# Autodesk Inventor assembly: Grundplatte_test
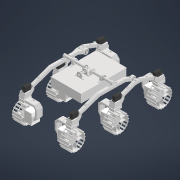
[picture p0: Inventor's stored thumbnail of the model, 180x180]
Saved by Autodesk Inventor 2021 (Build 250183000, 183)
## iProperties
Created: 2021-01-26
Part Number: Grundplatte_test
Document SubType Name: Assembly
Designer: Ctroi
Author: Ctroi
## Documents named in this file (33)
- G:\Roverprojekt\Github Projekt\Rover\Grundplatte_test.iam
- G:\Roverprojekt\Github Projekt\Rover\Grundplatte_hinten.ipt
- G:\Roverprojekt\Github Projekt\Rover\Grundplatte_vorne.ipt
- G:\Roverprojekt\Github Projekt\Rover\ArduinoMega.ipt
- G:\Roverprojekt\Github Projekt\Rover\Relais.ipt
- G:\Roverprojekt\Github Projekt\Rover\Kreuz_Halterung.ipt
- G:\Roverprojekt\Github Projekt\Rover\Obenplatte_hinten.ipt
- G:\Roverprojekt\Github Projekt\Rover\Obenplatte_vorne.ipt
- G:\Roverprojekt\Github Projekt\Rover\Halterung_Differential_3.ipt
- G:\Roverprojekt\Github Projekt\Rover\Halterung_Differential_Mitte.ipt
- G:\Roverprojekt\Github Projekt\Rover\Halterung_Differential.ipt
- G:\Roverprojekt\Github Projekt\Rover\Halterung_Differential_2.ipt
- G:\Roverprojekt\Github Projekt\Rover\Kugellager.ipt
- G:\Roverprojekt\Github Projekt\Rover\Kugellager_klein.ipt
- G:\Roverprojekt\Github Projekt\Rover\Verbindung_Rocker_Body.ipt
- G:\Roverprojekt\Github Projekt\Rover\Welle_Kugellager_Mitte.ipt
- G:\Roverprojekt\Github Projekt\Rover\Rocker_hinten_rechts.ipt
- G:\Roverprojekt\Github Projekt\Rover\Rocker_hinten.ipt
- G:\Roverprojekt\Github Projekt\Rover\Rocker_vorne.ipt
- G:\Roverprojekt\Github Projekt\Rover\Bogie.ipt
- G:\Roverprojekt\Github Projekt\Rover\Boogie_Stange.ipt
- G:\Roverprojekt\Github Projekt\Rover\Servohalterung_v2.ipt
- G:\Roverprojekt\Github Projekt\Rover\Servo.ipt
- G:\Roverprojekt\Github Projekt\Rover\Gegenstück_Welle_Diff.ipt
- G:\Roverprojekt\Github Projekt\Rover\Zahnrad_innen.ipt
- G:\Roverprojekt\Github Projekt\Rover\Übersetzungsbox_2.ipt
- G:\Roverprojekt\Github Projekt\Rover\Zahnrad_außen.ipt
- G:\Roverprojekt\Github Projekt\Rover\Motor_Servo_Welle_Test.ipt
- G:\Roverprojekt\Github Projekt\Rover\Verbindung_Motor_Servo_v2.ipt
- G:\Roverprojekt\Github Projekt\Rover\Motorhalterung_Klemme.ipt
- G:\Roverprojekt\Github Projekt\Rover\Motorhalterung_v2.ipt
- G:\Roverprojekt\Github Projekt\Rover\Steppermotor.ipt
- G:\Roverprojekt\Github Projekt\Rover\Reifen_v2.ipt
## Components (107 placed, 31 different names)
1. Grundplatte_hinten:1 — Passend:1, Passend:2, Passend:5, Passend:6, Passend:7, Passend:11, Passend:12, Passend:13, Passend:16
2. Grundplatte_vorne:1 — Passend:1, Passend:2, Passend:3, Passend:4, Passend:8, Passend:9, Passend:10, Passend:16
3. ArduinoMega:1 — Passend:3, Passend:4
4. Relais:1
5. Kreuz_Halterung:1 — Passend:5, Passend:6, Passend:7
6. Gegenstück_Welle_Diff:1 — Passend:96, Passend:97
7. Welle_Kugellager_Mitte:1 — Passend:48, Passend:49, Passend:96, Passend:97
8. Obenplatte_vorne:1 — Passend:8, Passend:9, Passend:10, Passend:15, Passend:17, Passend:18, Passend:21, Passend:22, Passend:23, Passend:24, Passend:27, Passend:28
9. Halterung_Differential_3:1 — Passend:14, Passend:15, Passend:17, Passend:38, Passend:39
10. Halterung_Differential_3:2 — Passend:18, Passend:19, Passend:20, Passend:32, Passend:33
11. Obenplatte_hinten:1 — Passend:11, Passend:12, Passend:13, Passend:14, Passend:19, Passend:20, Passend:25, Passend:26
12. Halterung_Differential_Mitte:1 — Passend:21, Passend:22, Passend:23, Passend:42, Passend:43
13. Halterung_Differential:1 — Passend:26, Passend:27, Passend:28, Passend:30, Passend:31, Passend:36, Passend:37
14. Halterung_Differential:2 — Passend:24, Passend:25, Passend:29, Passend:34, Passend:35
15. Halterung_Differential_2:1 — Passend:29, Passend:30, Passend:31, Passend:40, Passend:41
16. Kugellager:1 — Passend:40, Passend:41, Passend:48, Passend:49
17. Kugellager:2 — Passend:32, Passend:33, Passend:47
18. Kugellager:3 — Passend:34, Passend:35, Passend:44
19. Kugellager:4 — Passend:36, Passend:37, Passend:45
20. Kugellager:5 — Passend:38, Passend:39, Passend:46
21. Kugellager_klein:1 — Passend:42, Passend:43
22. Reifen_v2:6 — Einfügen:3
23. Reifen_v2:5 — Einfügen:4
24. Reifen_v2:4 — Einfügen:5
25. Steppermotor:6 — Passend:191, Passend:192, Passend:193, Einfügen:5
26. Steppermotor:5 — Passend:188, Passend:189, Passend:190, Einfügen:4
27. Steppermotor:4 — Passend:185, Passend:186, Passend:187, Einfügen:3
28. Motorhalterung_v2:3 — Fluchtend:41, Fluchtend:42, Passend:170, Passend:185, Passend:186, Passend:187
29. Motorhalterung_v2:2 — Fluchtend:43, Fluchtend:44, Passend:171, Passend:188, Passend:189, Passend:190
30. Motorhalterung_v2:1 — Fluchtend:45, Fluchtend:46, Passend:172, Passend:191, Passend:192, Passend:193
31. Motorhalterung_Klemme:3 — Fluchtend:33, Fluchtend:34, Passend:166, Fluchtend:45, Fluchtend:46, Passend:172
32. Motorhalterung_Klemme:2 — Fluchtend:31, Fluchtend:32, Passend:165, Fluchtend:43, Fluchtend:44, Passend:171
33. Motorhalterung_Klemme:1 — Fluchtend:29, Fluchtend:30, Passend:164, Fluchtend:41, Fluchtend:42, Passend:170
34. Verbindung_Motor_Servo_v2:6 — Passend:158, Passend:159, Fluchtend:29, Fluchtend:30, Passend:164
35. Verbindung_Motor_Servo_v2:5 — Passend:162, Passend:163, Fluchtend:33, Fluchtend:34, Passend:166
36. Verbindung_Motor_Servo_v2:4 — Passend:160, Passend:161, Fluchtend:31, Fluchtend:32, Passend:165
37. Motor_Servo_Welle_Test:6 — Passend:150, Passend:151, Passend:158, Passend:159
38. Motor_Servo_Welle_Test:5 — Passend:148, Passend:149, Passend:162, Passend:163
39. Motor_Servo_Welle_Test:4 — Passend:146, Passend:147, Passend:160, Passend:161
40. Zahnrad_außen:6 — Passend:136, Passend:137
41. Zahnrad_außen:5 — Passend:138, Passend:139
42. Zahnrad_außen:4 — Passend:134, Passend:135
43. Kugellager:14 — Passend:122, Passend:123, Passend:148, Passend:149
44. Kugellager:13 — Passend:124, Passend:125, Passend:146, Passend:147
45. Kugellager:10 — Passend:126, Passend:127, Passend:150, Passend:151
46. Übersetzungsbox_2:6 — Fluchtend:25, Fluchtend:26, Passend:114, Passend:124, Passend:125
47. Übersetzungsbox_2:3 — Fluchtend:27, Fluchtend:28, Passend:115, Passend:122, Passend:123
48. Übersetzungsbox_2:2 — Fluchtend:19, Fluchtend:20, Passend:111, Passend:126, Passend:127
49. Zahnrad_innen:3 — Passend:102, Passend:103, Passend:136, Passend:137
50. Zahnrad_innen:2 — Passend:100, Passend:101, Passend:138, Passend:139
51. Zahnrad_innen:1 — Passend:98, Passend:99, Passend:134, Passend:135
52. Servo:3 — Passend:81, Passend:82, Passend:83, Passend:102, Passend:103
53. Servo:5 — Passend:93, Passend:94, Passend:95, Passend:100, Passend:101
54. Servo:2 — Passend:90, Passend:91, Passend:92, Passend:98, Passend:99
55. Servohalterung_v2:5 — Fluchtend:15, Fluchtend:16, Passend:77, Passend:90, Passend:91, Passend:92, Fluchtend:19, Fluchtend:20, Passend:111
56. Servohalterung_v2:3 — Fluchtend:13, Fluchtend:14, Passend:76, Passend:93, Passend:94, Passend:95, Fluchtend:25, Fluchtend:26, Passend:114
57. Servohalterung_v2:2 — Fluchtend:11, Fluchtend:12, Passend:75, Passend:81, Passend:82, Passend:83, Fluchtend:27, Fluchtend:28, Passend:115
58. Boogie_Stange:1 — Passend:64, Passend:65, Passend:68, Passend:69
59. Fahrwerk_bogie:2 — Passend:68, Passend:69, Fluchtend:13, Fluchtend:14, Passend:76, Fluchtend:15, Fluchtend:16, Passend:77
60. Fahrwerk_rocker_vorne:1 — Fluchtend:1, Fluchtend:2, Passend:62, Fluchtend:11, Fluchtend:12, Passend:75
61. Kugellager:7 — Passend:54, Passend:55, Passend:64, Passend:65
62. Kugellager:6 — Passend:52, Passend:53
63. Fahrwerk_rocker_hinten:1 — Passend:50, Passend:51, Passend:52, Passend:53, Passend:54, Passend:55, Fluchtend:1, Fluchtend:2, Passend:62
64. Verbindung_Rocker_Body:1 — Passend:44, Passend:47, Passend:50, Passend:51
65. Reifen_v2:3 — Einfügen:2
66. Reifen_v2:2 — Einfügen:1
67. Reifen_v2:1
68. Steppermotor:3 — Passend:182, Passend:183, Passend:184
69. Steppermotor:2 — Passend:179, Passend:180, Passend:181, Einfügen:2
70. Steppermotor:1 — Passend:176, Passend:177, Passend:178, Einfügen:1
71. Motorhalterung_v2:6 — Fluchtend:51, Fluchtend:52, Passend:175, Passend:182, Passend:183, Passend:184
72. Motorhalterung_v2:5 — Fluchtend:49, Fluchtend:50, Passend:174, Passend:179, Passend:180, Passend:181
73. Motorhalterung_v2:4 — Fluchtend:47, Fluchtend:48, Passend:173, Passend:176, Passend:177, Passend:178
74. Motorhalterung_Klemme:4 — Fluchtend:35, Fluchtend:36, Passend:167, Fluchtend:47, Fluchtend:48, Passend:173
75. Motorhalterung_Klemme:5 — Fluchtend:37, Fluchtend:38, Passend:168, Fluchtend:49, Fluchtend:50, Passend:174
76. Motorhalterung_Klemme:6 — Fluchtend:39, Fluchtend:40, Passend:169, Fluchtend:51, Fluchtend:52, Passend:175
77. Verbindung_Motor_Servo_v2:3 — Passend:152, Passend:153, Fluchtend:35, Fluchtend:36, Passend:167
78. Verbindung_Motor_Servo_v2:2 — Passend:156, Passend:157, Fluchtend:39, Fluchtend:40, Passend:169
79. Verbindung_Motor_Servo_v2:1 — Passend:154, Passend:155, Fluchtend:37, Fluchtend:38, Passend:168
80. Motor_Servo_Welle_Test:3 — Passend:144, Passend:145, Passend:156, Passend:157
81. Motor_Servo_Welle_Test:2 — Passend:140, Passend:141, Passend:152, Passend:153
82. Motor_Servo_Welle_Test:1 — Passend:142, Passend:143, Passend:154, Passend:155
83. Zahnrad_außen:3 — Passend:132, Passend:133
84. Zahnrad_außen:2 — Passend:130, Passend:131
85. Zahnrad_außen:1 — Passend:128, Passend:129
86. Kugellager:15 — Passend:120, Passend:121, Passend:140, Passend:141
87. Kugellager:12 — Passend:118, Passend:119, Passend:142, Passend:143
88. Kugellager:11 — Passend:116, Passend:117, Passend:144, Passend:145
89. Übersetzungsbox_2:5 — Fluchtend:21, Fluchtend:22, Passend:112, Passend:118, Passend:119
90. Übersetzungsbox_2:4 — Fluchtend:23, Fluchtend:24, Passend:113, Passend:120, Passend:121
91. Übersetzungsbox_2:1 — Fluchtend:17, Fluchtend:18, Passend:110, Passend:116, Passend:117
92. Zahnrad_innen:6 — Passend:108, Passend:109, Passend:132, Passend:133
93. Zahnrad_innen:5 — Passend:106, Passend:107, Passend:130, Passend:131
94. Zahnrad_innen:4 — Passend:104, Passend:105, Passend:128, Passend:129
95. Servo:4 — Passend:78, Passend:79, Passend:80, Passend:108, Passend:109
96. Servo:6 — Passend:84, Passend:85, Passend:86, Passend:106, Passend:107
97. Servo:1 — Passend:87, Passend:88, Passend:89, Passend:104, Passend:105
98. Servohalterung_v2:6 — Fluchtend:5, Fluchtend:6, Passend:72, Passend:87, Passend:88, Passend:89, Fluchtend:17, Fluchtend:18, Passend:110
99. Servohalterung_v2:4 — Fluchtend:7, Fluchtend:8, Passend:73, Passend:84, Passend:85, Passend:86, Fluchtend:21, Fluchtend:22, Passend:112
100. Servohalterung_v2:1 — Fluchtend:9, Fluchtend:10, Passend:74, Passend:78, Passend:79, Passend:80, Fluchtend:23, Fluchtend:24, Passend:113
101. Boogie_Stange:2 — Passend:66, Passend:67, Passend:70, Passend:71
102. Fahrwerk_bogie:1 — Passend:70, Passend:71, Fluchtend:5, Fluchtend:6, Passend:72, Fluchtend:7, Fluchtend:8, Passend:73
103. Kugellager:9 — Passend:60, Passend:61
104. Kugellager:8 — Passend:58, Passend:59, Passend:66, Passend:67
105. Fahrwerk_rocker_hinten:2 — Passend:56, Passend:57, Passend:58, Passend:59, Passend:60, Passend:61, Fluchtend:3, Fluchtend:4, Passend:63
106. Fahrwerk_rocker_vorne:2 — Fluchtend:3, Fluchtend:4, Passend:63, Fluchtend:9, Fluchtend:10, Passend:74
107. Verbindung_Rocker_Body:2 — Passend:45, Passend:46, Passend:56, Passend:57
## Relationships (250: Mate 193, Flush 52, Insert 5)
- Passend:1 [Mate]: Grundplatte_hinten:1 ↔ Grundplatte_vorne:1
- Passend:2 [Mate]: Grundplatte_hinten:1 ↔ Grundplatte_vorne:1
- Passend:3 [Mate]: Grundplatte_vorne:1 ↔ ArduinoMega:1
- Passend:4 [Mate]: Grundplatte_vorne:1 ↔ ArduinoMega:1
- Passend:5 [Mate]: Grundplatte_hinten:1 ↔ Kreuz_Halterung:1
- Passend:6 [Mate]: Grundplatte_hinten:1 ↔ Kreuz_Halterung:1
- Passend:7 [Mate]: Grundplatte_hinten:1 ↔ Kreuz_Halterung:1
- Passend:8 [Mate]: Grundplatte_vorne:1 ↔ Obenplatte_vorne:1
- Passend:9 [Mate]: Grundplatte_vorne:1 ↔ Obenplatte_vorne:1
- Passend:10 [Mate]: Grundplatte_vorne:1 ↔ Obenplatte_vorne:1
- Passend:11 [Mate]: Grundplatte_hinten:1 ↔ Obenplatte_hinten:1
- Passend:12 [Mate]: Grundplatte_hinten:1 ↔ Obenplatte_hinten:1
- Passend:13 [Mate]: Grundplatte_hinten:1 ↔ Obenplatte_hinten:1
- Passend:14 [Mate]: Halterung_Differential_3:1 ↔ Obenplatte_hinten:1
- Passend:15 [Mate]: Obenplatte_vorne:1 ↔ Halterung_Differential_3:1
- Passend:16 [Mate]: Grundplatte_hinten:1 ↔ Grundplatte_vorne:1
- Passend:17 [Mate]: Obenplatte_vorne:1 ↔ Halterung_Differential_3:1
- Passend:18 [Mate]: Obenplatte_vorne:1 ↔ Halterung_Differential_3:2
- Passend:19 [Mate]: Halterung_Differential_3:2 ↔ Obenplatte_hinten:1
- Passend:20 [Mate]: Halterung_Differential_3:2 ↔ Obenplatte_hinten:1
- Passend:21 [Mate]: Obenplatte_vorne:1 ↔ Halterung_Differential_Mitte:1
- Passend:22 [Mate]: Obenplatte_vorne:1 ↔ Halterung_Differential_Mitte:1
- Passend:23 [Mate]: Obenplatte_vorne:1 ↔ Halterung_Differential_Mitte:1
- Passend:24 [Mate]: Obenplatte_vorne:1 ↔ Halterung_Differential:2
- Passend:25 [Mate]: Obenplatte_hinten:1 ↔ Halterung_Differential:2
- Passend:26 [Mate]: Obenplatte_hinten:1 ↔ Halterung_Differential:1
- Passend:27 [Mate]: Obenplatte_vorne:1 ↔ Halterung_Differential:1
- Passend:28 [Mate]: Obenplatte_vorne:1 ↔ Halterung_Differential:1
- Passend:29 [Mate]: Halterung_Differential:2 ↔ Halterung_Differential_2:1
- Passend:30 [Mate]: Halterung_Differential:1 ↔ Halterung_Differential_2:1
- Passend:31 [Mate]: Halterung_Differential:1 ↔ Halterung_Differential_2:1
- Passend:32 [Mate]: Halterung_Differential_3:2 ↔ Kugellager:2
- Passend:33 [Mate]: Halterung_Differential_3:2 ↔ Kugellager:2
- Passend:34 [Mate]: Halterung_Differential:2 ↔ Kugellager:3
- Passend:35 [Mate]: Halterung_Differential:2 ↔ Kugellager:3
- Passend:36 [Mate]: Halterung_Differential:1 ↔ Kugellager:4
- Passend:37 [Mate]: Halterung_Differential:1 ↔ Kugellager:4
- Passend:38 [Mate]: Halterung_Differential_3:1 ↔ Kugellager:5
- Passend:39 [Mate]: Halterung_Differential_3:1 ↔ Kugellager:5
- Passend:40 [Mate]: Halterung_Differential_2:1 ↔ Kugellager:1
- Passend:41 [Mate]: Halterung_Differential_2:1 ↔ Kugellager:1
- Passend:42 [Mate]: Halterung_Differential_Mitte:1 ↔ Kugellager_klein:1
- Passend:43 [Mate]: Halterung_Differential_Mitte:1 ↔ Kugellager_klein:1
- Passend:44 [Mate]: Kugellager:3 ↔ Verbindung_Rocker_Body:1
- Passend:45 [Mate]: Kugellager:4 ↔ Verbindung_Rocker_Body:2
- Passend:46 [Mate]: Kugellager:5 ↔ Verbindung_Rocker_Body:2
- Passend:47 [Mate]: Kugellager:2 ↔ Verbindung_Rocker_Body:1
- Passend:48 [Mate]: Welle_Kugellager_Mitte:1 ↔ Kugellager:1
- Passend:49 [Mate]: Welle_Kugellager_Mitte:1 ↔ Kugellager:1
- Passend:50 [Mate]: Fahrwerk_rocker_hinten:1 ↔ Verbindung_Rocker_Body:1
- Passend:51 [Mate]: Fahrwerk_rocker_hinten:1 ↔ Verbindung_Rocker_Body:1
- Passend:52 [Mate]: Kugellager:6 ↔ Fahrwerk_rocker_hinten:1
- Passend:53 [Mate]: Kugellager:6 ↔ Fahrwerk_rocker_hinten:1
- Passend:54 [Mate]: Kugellager:7 ↔ Fahrwerk_rocker_hinten:1
- Passend:55 [Mate]: Kugellager:7 ↔ Fahrwerk_rocker_hinten:1
- Passend:56 [Mate]: Fahrwerk_rocker_hinten:2 ↔ Verbindung_Rocker_Body:2
- Passend:57 [Mate]: Fahrwerk_rocker_hinten:2 ↔ Verbindung_Rocker_Body:2
- Passend:58 [Mate]: Kugellager:8 ↔ Fahrwerk_rocker_hinten:2
- Passend:59 [Mate]: Kugellager:8 ↔ Fahrwerk_rocker_hinten:2
- Passend:60 [Mate]: Kugellager:9 ↔ Fahrwerk_rocker_hinten:2
- Passend:61 [Mate]: Kugellager:9 ↔ Fahrwerk_rocker_hinten:2
- Fluchtend:1 [Flush]: Fahrwerk_rocker_vorne:1 ↔ Fahrwerk_rocker_hinten:1
- Fluchtend:2 [Flush]: Fahrwerk_rocker_vorne:1 ↔ Fahrwerk_rocker_hinten:1
- Passend:62 [Mate]: Fahrwerk_rocker_vorne:1 ↔ Fahrwerk_rocker_hinten:1
- Fluchtend:3 [Flush]: Fahrwerk_rocker_hinten:2 ↔ Fahrwerk_rocker_vorne:2
- Fluchtend:4 [Flush]: Fahrwerk_rocker_hinten:2 ↔ Fahrwerk_rocker_vorne:2
- Passend:63 [Mate]: Fahrwerk_rocker_hinten:2 ↔ Fahrwerk_rocker_vorne:2
- Passend:64 [Mate]: Boogie_Stange:1 ↔ Kugellager:7
- Passend:65 [Mate]: Boogie_Stange:1 ↔ Kugellager:7
- Passend:66 [Mate]: Boogie_Stange:2 ↔ Kugellager:8
- Passend:67 [Mate]: Boogie_Stange:2 ↔ Kugellager:8
- Passend:68 [Mate]: Boogie_Stange:1 ↔ Fahrwerk_bogie:2
- Passend:69 [Mate]: Boogie_Stange:1 ↔ Fahrwerk_bogie:2
- Passend:70 [Mate]: Boogie_Stange:2 ↔ Fahrwerk_bogie:1
- Passend:71 [Mate]: Boogie_Stange:2 ↔ Fahrwerk_bogie:1
- Fluchtend:5 [Flush]: Servohalterung_v2:6 ↔ Fahrwerk_bogie:1
- Fluchtend:6 [Flush]: Servohalterung_v2:6 ↔ Fahrwerk_bogie:1
- Passend:72 [Mate]: Servohalterung_v2:6 ↔ Fahrwerk_bogie:1
- Fluchtend:7 [Flush]: Servohalterung_v2:4 ↔ Fahrwerk_bogie:1
- Fluchtend:8 [Flush]: Servohalterung_v2:4 ↔ Fahrwerk_bogie:1
- Passend:73 [Mate]: Servohalterung_v2:4 ↔ Fahrwerk_bogie:1
- Fluchtend:9 [Flush]: Servohalterung_v2:1 ↔ Fahrwerk_rocker_vorne:2
- Fluchtend:10 [Flush]: Servohalterung_v2:1 ↔ Fahrwerk_rocker_vorne:2
- Passend:74 [Mate]: Servohalterung_v2:1 ↔ Fahrwerk_rocker_vorne:2
- Fluchtend:11 [Flush]: Servohalterung_v2:2 ↔ Fahrwerk_rocker_vorne:1
- Fluchtend:12 [Flush]: Servohalterung_v2:2 ↔ Fahrwerk_rocker_vorne:1
- Passend:75 [Mate]: Servohalterung_v2:2 ↔ Fahrwerk_rocker_vorne:1
- Fluchtend:13 [Flush]: Servohalterung_v2:3 ↔ Fahrwerk_bogie:2
- Fluchtend:14 [Flush]: Servohalterung_v2:3 ↔ Fahrwerk_bogie:2
- Passend:76 [Mate]: Servohalterung_v2:3 ↔ Fahrwerk_bogie:2
- Fluchtend:15 [Flush]: Servohalterung_v2:5 ↔ Fahrwerk_bogie:2
- Fluchtend:16 [Flush]: Servohalterung_v2:5 ↔ Fahrwerk_bogie:2
- Passend:77 [Mate]: Servohalterung_v2:5 ↔ Fahrwerk_bogie:2
- Passend:78 [Mate]: Servo:4 ↔ Servohalterung_v2:1
- Passend:79 [Mate]: Servo:4 ↔ Servohalterung_v2:1
- Passend:80 [Mate]: Servo:4 ↔ Servohalterung_v2:1
- Passend:81 [Mate]: Servo:3 ↔ Servohalterung_v2:2
- Passend:82 [Mate]: Servo:3 ↔ Servohalterung_v2:2
- Passend:83 [Mate]: Servo:3 ↔ Servohalterung_v2:2
- Passend:84 [Mate]: Servo:6 ↔ Servohalterung_v2:4
- Passend:85 [Mate]: Servo:6 ↔ Servohalterung_v2:4
- Passend:86 [Mate]: Servo:6 ↔ Servohalterung_v2:4
- Passend:87 [Mate]: Servo:1 ↔ Servohalterung_v2:6
- Passend:88 [Mate]: Servo:1 ↔ Servohalterung_v2:6
- Passend:89 [Mate]: Servo:1 ↔ Servohalterung_v2:6
- Passend:90 [Mate]: Servo:2 ↔ Servohalterung_v2:5
- Passend:91 [Mate]: Servo:2 ↔ Servohalterung_v2:5
- Passend:92 [Mate]: Servo:2 ↔ Servohalterung_v2:5
- Passend:93 [Mate]: Servo:5 ↔ Servohalterung_v2:3
- Passend:94 [Mate]: Servo:5 ↔ Servohalterung_v2:3
- Passend:95 [Mate]: Servo:5 ↔ Servohalterung_v2:3
- Passend:96 [Mate]: Gegenstück_Welle_Diff:1 ↔ Welle_Kugellager_Mitte:1
- Passend:97 [Mate]: Gegenstück_Welle_Diff:1 ↔ Welle_Kugellager_Mitte:1
- Passend:98 [Mate]: Zahnrad_innen:1 ↔ Servo:2
- Passend:99 [Mate]: Zahnrad_innen:1 ↔ Servo:2
- Passend:100 [Mate]: Zahnrad_innen:2 ↔ Servo:5
- Passend:101 [Mate]: Zahnrad_innen:2 ↔ Servo:5
- Passend:102 [Mate]: Zahnrad_innen:3 ↔ Servo:3
- Passend:103 [Mate]: Zahnrad_innen:3 ↔ Servo:3
- Passend:104 [Mate]: Zahnrad_innen:4 ↔ Servo:1
- Passend:105 [Mate]: Zahnrad_innen:4 ↔ Servo:1
- Passend:106 [Mate]: Zahnrad_innen:5 ↔ Servo:6
- Passend:107 [Mate]: Zahnrad_innen:5 ↔ Servo:6
- Passend:108 [Mate]: Zahnrad_innen:6 ↔ Servo:4
- Passend:109 [Mate]: Zahnrad_innen:6 ↔ Servo:4
- Fluchtend:17 [Flush]: Übersetzungsbox_2:1 ↔ Servohalterung_v2:6
- Fluchtend:18 [Flush]: Übersetzungsbox_2:1 ↔ Servohalterung_v2:6
- Passend:110 [Mate]: Übersetzungsbox_2:1 ↔ Servohalterung_v2:6
- Fluchtend:19 [Flush]: Übersetzungsbox_2:2 ↔ Servohalterung_v2:5
- Fluchtend:20 [Flush]: Übersetzungsbox_2:2 ↔ Servohalterung_v2:5
- Passend:111 [Mate]: Übersetzungsbox_2:2 ↔ Servohalterung_v2:5
- Fluchtend:21 [Flush]: Übersetzungsbox_2:5 ↔ Servohalterung_v2:4
- Fluchtend:22 [Flush]: Übersetzungsbox_2:5 ↔ Servohalterung_v2:4
- Passend:112 [Mate]: Übersetzungsbox_2:5 ↔ Servohalterung_v2:4
- Fluchtend:23 [Flush]: Übersetzungsbox_2:4 ↔ Servohalterung_v2:1
- Fluchtend:24 [Flush]: Übersetzungsbox_2:4 ↔ Servohalterung_v2:1
- Passend:113 [Mate]: Übersetzungsbox_2:4 ↔ Servohalterung_v2:1
- Fluchtend:25 [Flush]: Übersetzungsbox_2:6 ↔ Servohalterung_v2:3
- Fluchtend:26 [Flush]: Übersetzungsbox_2:6 ↔ Servohalterung_v2:3
- Passend:114 [Mate]: Übersetzungsbox_2:6 ↔ Servohalterung_v2:3
- Fluchtend:27 [Flush]: Übersetzungsbox_2:3 ↔ Servohalterung_v2:2
- Fluchtend:28 [Flush]: Übersetzungsbox_2:3 ↔ Servohalterung_v2:2
- Passend:115 [Mate]: Übersetzungsbox_2:3 ↔ Servohalterung_v2:2
- Passend:116 [Mate]: Kugellager:11 ↔ Übersetzungsbox_2:1
- Passend:117 [Mate]: Kugellager:11 ↔ Übersetzungsbox_2:1
- Passend:118 [Mate]: Kugellager:12 ↔ Übersetzungsbox_2:5
- Passend:119 [Mate]: Kugellager:12 ↔ Übersetzungsbox_2:5
- Passend:120 [Mate]: Kugellager:15 ↔ Übersetzungsbox_2:4
- Passend:121 [Mate]: Kugellager:15 ↔ Übersetzungsbox_2:4
- Passend:122 [Mate]: Kugellager:14 ↔ Übersetzungsbox_2:3
- Passend:123 [Mate]: Kugellager:14 ↔ Übersetzungsbox_2:3
- Passend:124 [Mate]: Kugellager:13 ↔ Übersetzungsbox_2:6
- Passend:125 [Mate]: Kugellager:13 ↔ Übersetzungsbox_2:6
- Passend:126 [Mate]: Kugellager:10 ↔ Übersetzungsbox_2:2
- Passend:127 [Mate]: Kugellager:10 ↔ Übersetzungsbox_2:2
- Passend:128 [Mate]: Zahnrad_außen:1 ↔ Zahnrad_innen:4
- Passend:129 [Mate]: Zahnrad_außen:1 ↔ Zahnrad_innen:4
- Passend:130 [Mate]: Zahnrad_außen:2 ↔ Zahnrad_innen:5
- Passend:131 [Mate]: Zahnrad_außen:2 ↔ Zahnrad_innen:5
- Passend:132 [Mate]: Zahnrad_außen:3 ↔ Zahnrad_innen:6
- Passend:133 [Mate]: Zahnrad_außen:3 ↔ Zahnrad_innen:6
- Passend:134 [Mate]: Zahnrad_außen:4 ↔ Zahnrad_innen:1
- Passend:135 [Mate]: Zahnrad_außen:4 ↔ Zahnrad_innen:1
- Passend:136 [Mate]: Zahnrad_außen:6 ↔ Zahnrad_innen:3
- Passend:137 [Mate]: Zahnrad_außen:6 ↔ Zahnrad_innen:3
- Passend:138 [Mate]: Zahnrad_außen:5 ↔ Zahnrad_innen:2
- Passend:139 [Mate]: Zahnrad_außen:5 ↔ Zahnrad_innen:2
- Passend:140 [Mate]: Motor_Servo_Welle_Test:2 ↔ Kugellager:15
- Passend:141 [Mate]: Motor_Servo_Welle_Test:2 ↔ Kugellager:15
- Passend:142 [Mate]: Motor_Servo_Welle_Test:1 ↔ Kugellager:12
- Passend:143 [Mate]: Motor_Servo_Welle_Test:1 ↔ Kugellager:12
- Passend:144 [Mate]: Motor_Servo_Welle_Test:3 ↔ Kugellager:11
- Passend:145 [Mate]: Motor_Servo_Welle_Test:3 ↔ Kugellager:11
- Passend:146 [Mate]: Motor_Servo_Welle_Test:4 ↔ Kugellager:13
- Passend:147 [Mate]: Motor_Servo_Welle_Test:4 ↔ Kugellager:13
- Passend:148 [Mate]: Motor_Servo_Welle_Test:5 ↔ Kugellager:14
- Passend:149 [Mate]: Motor_Servo_Welle_Test:5 ↔ Kugellager:14
- Passend:150 [Mate]: Motor_Servo_Welle_Test:6 ↔ Kugellager:10
- Passend:151 [Mate]: Motor_Servo_Welle_Test:6 ↔ Kugellager:10
- Passend:152 [Mate]: Verbindung_Motor_Servo_v2:3 ↔ Motor_Servo_Welle_Test:2
- Passend:153 [Mate]: Verbindung_Motor_Servo_v2:3 ↔ Motor_Servo_Welle_Test:2
- Passend:154 [Mate]: Verbindung_Motor_Servo_v2:1 ↔ Motor_Servo_Welle_Test:1
- Passend:155 [Mate]: Verbindung_Motor_Servo_v2:1 ↔ Motor_Servo_Welle_Test:1
- Passend:156 [Mate]: Verbindung_Motor_Servo_v2:2 ↔ Motor_Servo_Welle_Test:3
- Passend:157 [Mate]: Verbindung_Motor_Servo_v2:2 ↔ Motor_Servo_Welle_Test:3
- Passend:158 [Mate]: Verbindung_Motor_Servo_v2:6 ↔ Motor_Servo_Welle_Test:6
- Passend:159 [Mate]: Verbindung_Motor_Servo_v2:6 ↔ Motor_Servo_Welle_Test:6
- Passend:160 [Mate]: Verbindung_Motor_Servo_v2:4 ↔ Motor_Servo_Welle_Test:4
- Passend:161 [Mate]: Verbindung_Motor_Servo_v2:4 ↔ Motor_Servo_Welle_Test:4
- Passend:162 [Mate]: Verbindung_Motor_Servo_v2:5 ↔ Motor_Servo_Welle_Test:5
- Passend:163 [Mate]: Verbindung_Motor_Servo_v2:5 ↔ Motor_Servo_Welle_Test:5
- Fluchtend:29 [Flush]: Motorhalterung_Klemme:1 ↔ Verbindung_Motor_Servo_v2:6
- Fluchtend:30 [Flush]: Motorhalterung_Klemme:1 ↔ Verbindung_Motor_Servo_v2:6
- Passend:164 [Mate]: Motorhalterung_Klemme:1 ↔ Verbindung_Motor_Servo_v2:6
- Fluchtend:31 [Flush]: Motorhalterung_Klemme:2 ↔ Verbindung_Motor_Servo_v2:4
- Fluchtend:32 [Flush]: Motorhalterung_Klemme:2 ↔ Verbindung_Motor_Servo_v2:4
- Passend:165 [Mate]: Motorhalterung_Klemme:2 ↔ Verbindung_Motor_Servo_v2:4
- Fluchtend:33 [Flush]: Motorhalterung_Klemme:3 ↔ Verbindung_Motor_Servo_v2:5
- Fluchtend:34 [Flush]: Motorhalterung_Klemme:3 ↔ Verbindung_Motor_Servo_v2:5
- Passend:166 [Mate]: Motorhalterung_Klemme:3 ↔ Verbindung_Motor_Servo_v2:5
- Fluchtend:35 [Flush]: Motorhalterung_Klemme:4 ↔ Verbindung_Motor_Servo_v2:3
- Fluchtend:36 [Flush]: Motorhalterung_Klemme:4 ↔ Verbindung_Motor_Servo_v2:3
- Passend:167 [Mate]: Motorhalterung_Klemme:4 ↔ Verbindung_Motor_Servo_v2:3
- Fluchtend:37 [Flush]: Motorhalterung_Klemme:5 ↔ Verbindung_Motor_Servo_v2:1
- Fluchtend:38 [Flush]: Motorhalterung_Klemme:5 ↔ Verbindung_Motor_Servo_v2:1
- Passend:168 [Mate]: Motorhalterung_Klemme:5 ↔ Verbindung_Motor_Servo_v2:1
- Fluchtend:39 [Flush]: Motorhalterung_Klemme:6 ↔ Verbindung_Motor_Servo_v2:2
- Fluchtend:40 [Flush]: Motorhalterung_Klemme:6 ↔ Verbindung_Motor_Servo_v2:2
- Passend:169 [Mate]: Motorhalterung_Klemme:6 ↔ Verbindung_Motor_Servo_v2:2
- Fluchtend:41 [Flush]: Motorhalterung_v2:3 ↔ Motorhalterung_Klemme:1
- Fluchtend:42 [Flush]: Motorhalterung_v2:3 ↔ Motorhalterung_Klemme:1
- Passend:170 [Mate]: Motorhalterung_v2:3 ↔ Motorhalterung_Klemme:1
- Fluchtend:43 [Flush]: Motorhalterung_v2:2 ↔ Motorhalterung_Klemme:2
- Fluchtend:44 [Flush]: Motorhalterung_v2:2 ↔ Motorhalterung_Klemme:2
- Passend:171 [Mate]: Motorhalterung_v2:2 ↔ Motorhalterung_Klemme:2
- Fluchtend:45 [Flush]: Motorhalterung_v2:1 ↔ Motorhalterung_Klemme:3
- Fluchtend:46 [Flush]: Motorhalterung_v2:1 ↔ Motorhalterung_Klemme:3
- Passend:172 [Mate]: Motorhalterung_v2:1 ↔ Motorhalterung_Klemme:3
- Fluchtend:47 [Flush]: Motorhalterung_v2:4 ↔ Motorhalterung_Klemme:4
- Fluchtend:48 [Flush]: Motorhalterung_v2:4 ↔ Motorhalterung_Klemme:4
- Passend:173 [Mate]: Motorhalterung_v2:4 ↔ Motorhalterung_Klemme:4
- Fluchtend:49 [Flush]: Motorhalterung_v2:5 ↔ Motorhalterung_Klemme:5
- Fluchtend:50 [Flush]: Motorhalterung_v2:5 ↔ Motorhalterung_Klemme:5
- Passend:174 [Mate]: Motorhalterung_v2:5 ↔ Motorhalterung_Klemme:5
- Fluchtend:51 [Flush]: Motorhalterung_v2:6 ↔ Motorhalterung_Klemme:6
- Fluchtend:52 [Flush]: Motorhalterung_v2:6 ↔ Motorhalterung_Klemme:6
- Passend:175 [Mate]: Motorhalterung_v2:6 ↔ Motorhalterung_Klemme:6
- Passend:176 [Mate]: Steppermotor:1 ↔ Motorhalterung_v2:4
- Passend:177 [Mate]: Steppermotor:1 ↔ Motorhalterung_v2:4
- Passend:178 [Mate]: Steppermotor:1 ↔ Motorhalterung_v2:4
- Passend:179 [Mate]: Steppermotor:2 ↔ Motorhalterung_v2:5
- Passend:180 [Mate]: Steppermotor:2 ↔ Motorhalterung_v2:5
- Passend:181 [Mate]: Steppermotor:2 ↔ Motorhalterung_v2:5
- Passend:182 [Mate]: Steppermotor:3 ↔ Motorhalterung_v2:6
- Passend:183 [Mate]: Steppermotor:3 ↔ Motorhalterung_v2:6
- Passend:184 [Mate]: Steppermotor:3 ↔ Motorhalterung_v2:6
- Passend:185 [Mate]: Steppermotor:4 ↔ Motorhalterung_v2:3
- Passend:186 [Mate]: Steppermotor:4 ↔ Motorhalterung_v2:3
- Passend:187 [Mate]: Steppermotor:4 ↔ Motorhalterung_v2:3
- Passend:188 [Mate]: Steppermotor:5 ↔ Motorhalterung_v2:2
- Passend:189 [Mate]: Steppermotor:5 ↔ Motorhalterung_v2:2
- Passend:190 [Mate]: Steppermotor:5 ↔ Motorhalterung_v2:2
- Passend:191 [Mate]: Steppermotor:6 ↔ Motorhalterung_v2:1
- Passend:192 [Mate]: Steppermotor:6 ↔ Motorhalterung_v2:1
- Passend:193 [Mate]: Steppermotor:6 ↔ Motorhalterung_v2:1
- Einfügen:1 [Insert] (-15 mm): Reifen_v2:2 ↔ Steppermotor:1
- Einfügen:2 [Insert] (-15 mm): Reifen_v2:3 ↔ Steppermotor:2
- Einfügen:3 [Insert] (-15 mm): Reifen_v2:6 ↔ Steppermotor:4
- Einfügen:4 [Insert] (-15 mm): Reifen_v2:5 ↔ Steppermotor:5
- Einfügen:5 [Insert] (-15 mm): Reifen_v2:4 ↔ Steppermotor:6
